# Autodesk Inventor assembly: Assembly bottom
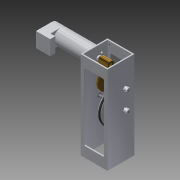
[picture p0: Inventor's stored thumbnail of the model, 180x180]
Saved by Autodesk Inventor 2015 (Build 190159000, 159)
## iProperties
Created: 2015-05-23
Part Number: Assembly bottom
Document SubType Name: Assembly
Designer: kenta
Mass: 273.543 g
Surface Area: 574.77 cm^2
Volume: 81.5679 cm^3
Density: 3.35357 g/cm^3
Author: kenta
## Documents named in this file (12)
- C:\Users\kenta\Documents\Inventor\知能ロボコン\Assembly bottom.iam
- C:\Users\kenta\Documents\Inventor\知能ロボコン\Gear box.ipt
- C:\Users\kenta\Documents\Inventor\知能ロボコン\Gear1_BSS0.5-20B.ipt
- C:\Users\kenta\Documents\Inventor\知能ロボコン\Shaft.ipt
- C:\Users\kenta\Documents\Inventor\知能ロボコン\Motor_A-max22.ipt
- C:\Users\kenta\Documents\Inventor\知能ロボコン\Bearing_SMF63ZZ.ipt
- C:\Users\kenta\Documents\Inventor\知能ロボコン\Wheel.ipt
- C:\Users\kenta\Documents\Inventor\知能ロボコン\Gear2_S50B 60B+0203.ipt
- C:\Users\kenta\Documents\Inventor\知能ロボコン\Gear3_S50B 30B+0303.ipt
- C:\Users\kenta\Documents\Inventor\知能ロボコン\Wheel ring.ipt
- C:\Users\kenta\Documents\Inventor\知能ロボコン\Stopper.ipt
- C:\Users\kenta\Documents\Inventor\知能ロボコン\Gear4_S50B 80B+0203.ipt
## Components (18 placed, 11 different names)
1. Gear box:1 — 挿入:1, 挿入:2, 挿入:3, 挿入:4, 挿入:5, 挿入:6, 挿入:10, 挿入:13
2. Gear1_BSS0.5-20B:1 — 挿入:7
3. Gear2_S50B 60B+0203:1 — 挿入:10, 挿入:14
4. Gear3_S50B 30B+0303:1 — 挿入:14
5. Wheel:1 — 挿入:13, メイト:1, 挿入:22
6. Bearing_SMF63ZZ:1 — 挿入:3, 挿入:8, 挿入:21
7. Bearing_SMF63ZZ:2 — 挿入:4, 挿入:20
8. Bearing_SMF63ZZ:3 — 挿入:5, 挿入:19
9. Bearing_SMF63ZZ:4 — 挿入:6, 挿入:9, 挿入:18
10. Shaft:1 — 挿入:8
11. Shaft:2 — 挿入:9
12. Motor_A-max22:1 — 挿入:1, 挿入:2, 挿入:7
13. Wheel ring:1 — メイト:1
14. Stopper:3 — 挿入:18
15. Stopper:4 — 挿入:20
16. Stopper:5 — 挿入:19
17. Stopper:6 — 挿入:21
18. Gear4_S50B 80B+0203:1 — 挿入:22
## Relationships (18: Insert 17, Mate 1)
- 挿入:1 [Insert]: Gear box:1 ↔ Motor_A-max22:1
- 挿入:2 [Insert]: Gear box:1 ↔ Motor_A-max22:1
- 挿入:3 [Insert]: Gear box:1 ↔ Bearing_SMF63ZZ:1
- 挿入:4 [Insert]: Gear box:1 ↔ Bearing_SMF63ZZ:2
- 挿入:5 [Insert]: Gear box:1 ↔ Bearing_SMF63ZZ:3
- 挿入:6 [Insert]: Gear box:1 ↔ Bearing_SMF63ZZ:4
- 挿入:7 [Insert] (2 mm): Gear1_BSS0.5-20B:1 ↔ Motor_A-max22:1
- 挿入:8 [Insert] (-5 mm): Bearing_SMF63ZZ:1 ↔ Shaft:1
- 挿入:9 [Insert] (-5 mm): Bearing_SMF63ZZ:4 ↔ Shaft:2
- 挿入:10 [Insert] (5.5 mm): Gear box:1 ↔ Gear2_S50B 60B+0203:1
- 挿入:13 [Insert] (9.5 mm): Gear box:1 ↔ Wheel:1
- 挿入:14 [Insert]: Gear2_S50B 60B+0203:1 ↔ Gear3_S50B 30B+0303:1
- メイト:1 [Mate]: Wheel:1 ↔ Wheel ring:1
- 挿入:18 [Insert]: Bearing_SMF63ZZ:4 ↔ Stopper:3
- 挿入:19 [Insert]: Bearing_SMF63ZZ:3 ↔ Stopper:5
- 挿入:20 [Insert]: Bearing_SMF63ZZ:2 ↔ Stopper:4
- 挿入:21 [Insert]: Bearing_SMF63ZZ:1 ↔ Stopper:6
- 挿入:22 [Insert]: Wheel:1 ↔ Gear4_S50B 80B+0203:1
